# Autodesk Inventor assembly: WheelDistances
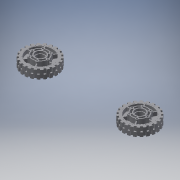
[picture p0: Inventor's stored thumbnail of the model, 180x180]
Saved by Autodesk Inventor 2016 SP1 (Build 200210100, 210)
## iProperties
Created: 2016-02-07
Part Number: WheelDistances
Document SubType Name: Assembly
Designer: steele
Author: steele
## Documents named in this file (2)
- C:\snobotics\CAD-Development\robSteele\SnoBotics2016\2016-05-05-ShooterPrototype\WheelDistances.iam
- C:\snobotics\CAD-Development\robSteele\SnoBotics2016\AM Parts\4 in HiGrip Wheel.iam
## Components (2 placed, 1 different names)
1. 4 in HiGrip Wheel:1 [sub-assembly] — Mate:1, Mate:2
2. 4 in HiGrip Wheel:2 [sub-assembly] — Mate:1, Mate:2
## Relationships (2: Mate 2)
- Mate:1: 4 in HiGrip Wheel:1 ↔ 4 in HiGrip Wheel:2
- Mate:2 (304.8 mm): 4 in HiGrip Wheel:1 ↔ 4 in HiGrip Wheel:2
